# Autodesk Inventor assembly: Rotrkopf
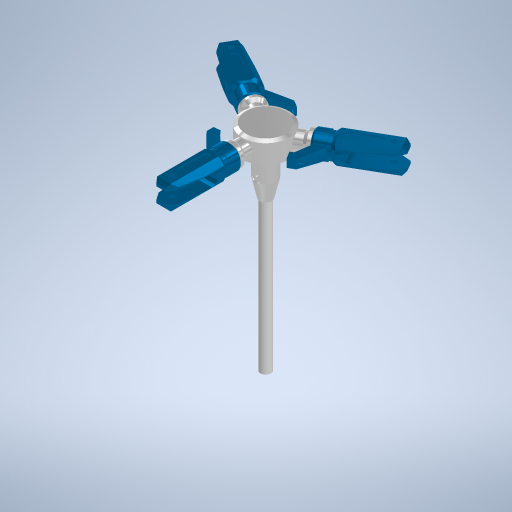
[picture p0: Inventor's stored thumbnail of the model, 512x512]
Saved by Autodesk Inventor 2023.2 (Build 272271000, 271)
## iProperties
Created: 2023-03-31
Part Number: Rotrkopf
Document SubType Name: Assembly
Designer: tadeu
Author: tadeu
## Documents named in this file (4)
- C:\Users\tadeu\Documents\0 Nerdy\CAD\Inventor\Studium\5. Semester\NWPL\WKA\Rotrkopf.iam
- C:\Users\tadeu\Documents\0 Nerdy\CAD\Inventor\Studium\5. Semester\NWPL\WKA\RotorKopf_Hub.ipt
- C:\Users\tadeu\Documents\0 Nerdy\CAD\Inventor\Studium\5. Semester\NWPL\WKA\RotorArm.ipt
- C:\Users\tadeu\Documents\0 Nerdy\CAD\Inventor\Studium\5. Semester\NWPL\WKA\Welle.ipt
## Components (5 placed, 3 different names)
1. Welle:1 — Drehbar:1
2. RotorKopf_Hub:1 — Drehbar:1, Drehbar:2
3. RotorArm:1 — Drehbar:2
4. RotorArm:2
5. RotorArm:3
## Component patterns: (3 elements, first: RotorArm:1)
## Relationships (2: RevoluteJoint 2)
- Drehbar:1 [RevoluteJoint]: Welle:1 ↔ RotorKopf_Hub:1
- Drehbar:2 [RevoluteJoint]: RotorKopf_Hub:1 ↔ RotorArm:1
